# Autodesk Inventor assembly: Masses
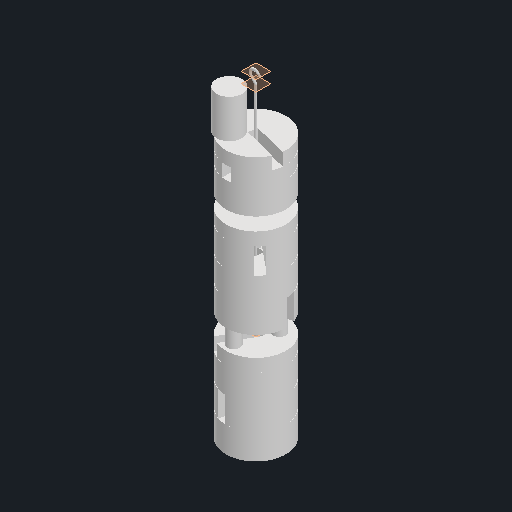
[picture p0: Inventor's stored thumbnail of the model, 512x512]
Saved by Autodesk Inventor 2023.1 (Build 271208000, 208)
## iProperties
Created: 2022-12-07
Part Number: Masses
Document SubType Name: Assembly
Designer: aubrey-work
Author: aubrey-work
## Documents named in this file (7)
- C:\GitHubRepos\PHYS-12-Website\content\portfolio\CAD Practice\Entries\3-Physics201L Test Hook Apparatus\Masses.iam
- C:\GitHubRepos\PHYS-12-Website\content\portfolio\CAD Practice\Entries\3-Physics201L Test Hook Apparatus\Double Hooked Mass.ipt
- C:\GitHubRepos\PHYS-12-Website\content\portfolio\CAD Practice\Entries\3-Physics201L Test Hook Apparatus\Long Hanging Mass 2.ipt
- C:\GitHubRepos\PHYS-12-Website\content\portfolio\CAD Practice\Entries\3-Physics201L Test Hook Apparatus\2kg Mass.ipt
- C:\GitHubRepos\PHYS-12-Website\content\portfolio\CAD Practice\Entries\3-Physics201L Test Hook Apparatus\1kg Disc Mass.ipt
- C:\GitHubRepos\PHYS-12-Website\content\portfolio\CAD Practice\Entries\3-Physics201L Test Hook Apparatus\50g Cylinder Standoff Mass.ipt
- C:\GitHubRepos\PHYS-12-Website\content\portfolio\CAD Practice\Entries\3-Physics201L Test Hook Apparatus\500g Cylinder Mass.ipt
## Components (17 placed, 6 different names)
1. Double Hooked Mass:1 — Mate:1, Flush:3, Flush:1, Mate:12, Mate:15, Mate:16, Mate:17, Mate:18, Mate:19, Mate:21, Mate:22
2. Long Hanging Mass 2:1 — Mate:1, Flush:3, Flush:1, Mate:2, Mate:3, Mate:5, Mate:6, Mate:8
3. 2kg Mass:1 — Mate:2, Mate:3, Mate:4
4. 1kg Disc Mass:1 — Mate:8, Mate:9, Mate:10, Mate:25, Mate:26
5. 50g Cylinder Standoff Mass:1 — Mate:10, Mate:11
6. 2kg Mass:2 — Mate:6, Mate:7, Mate:9
7. 2kg Mass:3 — Mate:4, Mate:5, Mate:7
8. 2kg Mass:4 — Mate:11, Mate:12, Mate:13
9. 2kg Mass:5 — Mate:13, Mate:14, Mate:18
10. 2kg Mass:6 — Mate:14, Mate:17, Mate:20
11. 2kg Mass:7 — Mate:15, Mate:16, Mate:23
12. 1kg Disc Mass:2 — Mate:19, Mate:20
13. 1kg Disc Mass:3 — Mate:21, Mate:23, Mate:24
14. 1kg Disc Mass:4 — Mate:22, Mate:24, Mate:27
15. 50g Cylinder Standoff Mass:2 — Mate:26
16. 50g Cylinder Standoff Mass:3 — Mate:25
17. 500g Cylinder Mass:1 — Mate:27
## Relationships (29: Mate 27, Flush 2)
- Mate:1: Double Hooked Mass:1 ↔ Long Hanging Mass 2:1
- Flush:3: Double Hooked Mass:1 ↔ Long Hanging Mass 2:1
- Flush:1: Double Hooked Mass:1 ↔ Long Hanging Mass 2:1
- Mate:2: Long Hanging Mass 2:1 ↔ 2kg Mass:1
- Mate:3: Long Hanging Mass 2:1 ↔ 2kg Mass:1
- Mate:4: 2kg Mass:1 ↔ 2kg Mass:3
- Mate:5: Long Hanging Mass 2:1 ↔ 2kg Mass:3
- Mate:6: Long Hanging Mass 2:1 ↔ 2kg Mass:2
- Mate:7: 2kg Mass:2 ↔ 2kg Mass:3
- Mate:8: Long Hanging Mass 2:1 ↔ 1kg Disc Mass:1
- Mate:9: 1kg Disc Mass:1 ↔ 2kg Mass:2
- Mate:10: 1kg Disc Mass:1 ↔ 50g Cylinder Standoff Mass:1
- Mate:11: 50g Cylinder Standoff Mass:1 ↔ 2kg Mass:4
- Mate:12: Double Hooked Mass:1 ↔ 2kg Mass:4
- Mate:13: 2kg Mass:4 ↔ 2kg Mass:5
- Mate:14: 2kg Mass:5 ↔ 2kg Mass:6
- Mate:15: Double Hooked Mass:1 ↔ 2kg Mass:7
- Mate:16: Double Hooked Mass:1 ↔ 2kg Mass:7
- Mate:17: Double Hooked Mass:1 ↔ 2kg Mass:6
- Mate:18: Double Hooked Mass:1 ↔ 2kg Mass:5
- Mate:19: Double Hooked Mass:1 ↔ 1kg Disc Mass:2
- Mate:20: 2kg Mass:6 ↔ 1kg Disc Mass:2
- Mate:21: Double Hooked Mass:1 ↔ 1kg Disc Mass:3
- Mate:22: Double Hooked Mass:1 ↔ 1kg Disc Mass:4
- Mate:23: 2kg Mass:7 ↔ 1kg Disc Mass:3
- Mate:24: 1kg Disc Mass:3 ↔ 1kg Disc Mass:4
- Mate:25: 1kg Disc Mass:1 ↔ 50g Cylinder Standoff Mass:3
- Mate:26: 1kg Disc Mass:1 ↔ 50g Cylinder Standoff Mass:2
- Mate:27: 1kg Disc Mass:4 ↔ 500g Cylinder Mass:1
